# Autodesk Inventor assembly: Assembly
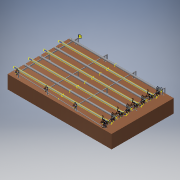
[picture p0: Inventor's stored thumbnail of the model, 180x180]
Saved by Autodesk Inventor 2017 (Build 210142000, 142)
## iProperties
Created: 2017-10-30
Part Number: Assembly
Document SubType Name: Assembly
Designer: DesignPC02
Author: DesignPC02
## Documents named in this file (19)
- C:\Users\DesignPC02\Desktop\hydroponic\Assembly.iam
- C:\Users\DesignPC02\Desktop\hydroponic\wall.ipt
- C:\Users\DesignPC02\Desktop\hydroponic\PipeA.ipt
- C:\Users\DesignPC02\Desktop\hydroponic\Stand.ipt
- C:\Users\DesignPC02\Desktop\hydroponic\PipeB.ipt
- C:\Users\DesignPC02\Desktop\hydroponic\Cap(right).ipt
- C:\Users\DesignPC02\Desktop\hydroponic\water setter.ipt
- C:\Users\DesignPC02\Desktop\hydroponic\90º Elbow.ipt
- C:\Users\DesignPC02\Desktop\hydroponic\Elbow and Tee conector.ipt
- C:\Users\DesignPC02\Desktop\hydroponic\Tee.ipt
- C:\Users\DesignPC02\Desktop\hydroponic\water out put.ipt
- C:\Users\DesignPC02\Desktop\hydroponic\Bottom pipe.ipt
- C:\Users\DesignPC02\Desktop\hydroponic\Cap(left).ipt
- C:\Users\DesignPC02\Desktop\hydroponic\Black part to elbow.ipt
- C:\Users\DesignPC02\Desktop\hydroponic\elbow to tee.ipt
- C:\Users\DesignPC02\Desktop\hydroponic\Small Cap.ipt
- C:\Users\DesignPC02\Desktop\hydroponic\Water input.ipt
- C:\Users\DesignPC02\Desktop\hydroponic\Small pie 8mm.ipt
- C:\Users\DesignPC02\Desktop\hydroponic\Hange.ipt
## Components (85 placed, 18 different names)
1. wall:1 — Mate:1, Flush:1, Mate:2, Mate:3, Mate:4, Flush:2, Mate:5, Mate:6, Mate:8, Mate:35, Tangent:2
2. Elbow and Tee conector:9 — Mate:36, Mate:37, Mate:38
3. 90º Elbow:9 — Mate:38, Mate:39, Mate:40
4. Bottom pipe:1 — Mate:39, Mate:40
5. elbow to tee:9 — Mate:46, Mate:47, Mate:48, Mate:49
6. Small Cap:1 — Mate:48, Mate:49
7. Water input:1 — Tangent:1, Flush:54, Tangent:2, Mate:50, Mate:51, Mate:52
8. Small Cap:2 — Mate:50
9. Small pie 8mm:1 — Mate:51
10. Hange:1 — Mate:52
11. Stand:1 — Mate:2, Mate:3, Mate:4, Flush:2, Mate:5, Mate:6, Mate:7, Mate:33, Mate:35, Tangent:1, Flush:54
12. Stand:2
13. Stand:3
14. Stand:4 — Mate:14
15. PipeA:1 — Mate:1, Flush:1, Mate:7, Mate:9, Mate:12, Mate:13
16. PipeB:1 — Mate:8, Flush:3, Mate:9
17. PipeA:2
18. PipeB:2
19. PipeA:3
20. PipeB:3
21. PipeA:4
22. PipeB:4
23. Cap(right):1 — Mate:12, Mate:13, Mate:14, Mate:41, Mate:42
24. Cap(right):2
25. Cap(right):3
26. Cap(right):4
27. Cap(right):5
28. Cap(right):6
29. Cap(right):7
30. Cap(right):8
31. Tee:1 — Mate:22, Mate:23, Mate:45, Mate:46, Mate:47
32. Tee:2
33. Tee:3
34. Tee:4
35. Tee:5
36. Tee:6
37. Tee:7
38. Tee:8 — Mate:36, Mate:37
39. water out put:1 — Mate:22, Mate:23
40. water out put:2
41. water out put:3
42. water out put:4
43. water out put:5
44. water out put:6
45. water out put:7
46. Cap(left):1 — Mate:33
47. Cap(left):2
48. Cap(left):3
49. Cap(left):4
50. Cap(left):5
51. Cap(left):6
52. Cap(left):7
53. Cap(left):8
54. water setter:1 — Mate:41, Mate:42, Mate:43
55. water setter:2
56. water setter:3
57. water setter:4
58. water setter:5
59. water setter:6
60. water setter:7
61. water setter:8
62. Black part to elbow:1 — Mate:43, Mate:44
63. Black part to elbow:2
64. Black part to elbow:3
65. Black part to elbow:4
66. Black part to elbow:5
67. Black part to elbow:6
68. Black part to elbow:7
69. Black part to elbow:8
70. 90º Elbow:10 — Mate:44
71. 90º Elbow:11
72. 90º Elbow:12
73. 90º Elbow:13
74. 90º Elbow:14
75. 90º Elbow:15
76. 90º Elbow:16
77. 90º Elbow:17
78. elbow to tee:1 — Mate:45
79. elbow to tee:2
80. elbow to tee:3
81. elbow to tee:4
82. elbow to tee:5
83. elbow to tee:6
84. elbow to tee:7
85. elbow to tee:8
## Component patterns: (4 elements, first: Stand:1), (4 elements, first: PipeA:1 + PipeB:1), (8 elements, first: Cap(right):1), (8 elements, first: Tee:1), (7 elements, first: water out put:1), (8 elements, first: Cap(left):1), (8 elements, first: water setter:1), (8 elements, first: Black part to elbow:1), (8 elements, first: 90º Elbow:10), (8 elements, first: elbow to tee:1)
## Relationships (39: Mate 33, Flush 4, Tangent 2)
- Mate:1 (267 mm): wall:1 ↔ PipeA:1
- Flush:1: wall:1 ↔ PipeA:1
- Mate:2: wall:1 ↔ Stand:1
- Mate:3: wall:1 ↔ Stand:1
- Mate:4: wall:1 ↔ Stand:1
- Flush:2 (-1964.5 mm): wall:1 ↔ Stand:1
- Mate:5: wall:1 ↔ Stand:1
- Mate:6: wall:1 ↔ Stand:1
- Mate:7: Stand:1 ↔ PipeA:1
- Mate:8 (267 mm): wall:1 ↔ PipeB:1
- Flush:3: PipeB:1
- Mate:9 (338 mm): PipeA:1 ↔ PipeB:1
- Mate:12: PipeA:1 ↔ Cap(right):1
- Mate:13: PipeA:1 ↔ Cap(right):1
- Mate:14 (18 mm): Stand:4 ↔ Cap(right):1
- Mate:22: Tee:1 ↔ water out put:1
- Mate:23 (119 mm): Tee:1 ↔ water out put:1
- Mate:33 (3 mm): Stand:1 ↔ Cap(left):1
- Mate:35: wall:1 ↔ Stand:1
- Mate:36: Elbow and Tee conector:9 ↔ Tee:8
- Mate:37: Elbow and Tee conector:9 ↔ Tee:8
- Mate:38: Elbow and Tee conector:9 ↔ 90º Elbow:9
- Mate:39: 90º Elbow:9 ↔ Bottom pipe:1
- Mate:40 (1975 mm): 90º Elbow:9 ↔ Bottom pipe:1
- Mate:41: Cap(right):1 ↔ water setter:1
- Mate:42 (-38 mm): Cap(right):1 ↔ water setter:1
- Mate:43: water setter:1 ↔ Black part to elbow:1
- Mate:44: Black part to elbow:1 ↔ 90º Elbow:10
- Mate:45: Tee:1 ↔ elbow to tee:1
- Mate:46 (16 mm): elbow to tee:9 ↔ Tee:1
- Mate:47: elbow to tee:9 ↔ Tee:1
- Mate:48: elbow to tee:9 ↔ Small Cap:1
- Mate:49: elbow to tee:9 ↔ Small Cap:1
- Tangent:1: Water input:1 ↔ Stand:1
- Flush:54: Water input:1 ↔ Stand:1
- Tangent:2 (150 mm): wall:1 ↔ Water input:1
- Mate:50: Water input:1 ↔ Small Cap:2
- Mate:51: Water input:1 ↔ Small pie 8mm:1
- Mate:52: Water input:1 ↔ Hange:1
